# Autodesk Inventor assembly: ForkMechanism_report
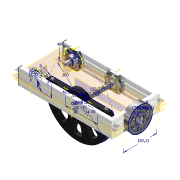
[picture p0: Inventor's stored thumbnail of the model, 180x180]
Saved by Autodesk Inventor 2022 (Build 260153000, 153)
## iProperties
Created: 2022-11-13
Part Number: ForkMechanism_report
Document SubType Name: Assembly
Designer: alexw
Author: alexw
## Documents named in this file (6)
- C:\Users\alexw\Documents\Inventor\Projects\03_CurrentProjects\MasterThesis\PSM_V1_Rillenkugellager\ForkMechanism_report.iam
- C:\Users\alexw\Documents\Inventor\Projects\03_CurrentProjects\MasterThesis\PSM_V1_Rillenkugellager\ParallelMecha_V2_BaseFrame_Item40x40.iam
- C:\Users\alexw\Documents\Inventor\Projects\03_CurrentProjects\MasterThesis\PSM_V1_Rillenkugellager\CapstonDisc_ParallelMecha.ipt
- C:\Users\alexw\Documents\Inventor\Projects\03_CurrentProjects\MasterThesis\PSM_V1_Rillenkugellager\ContentCenter\de-DE\ISO 4762(2)\ISO 4762 - M5 x 16ISO.ipt
- C:\Users\alexw\Documents\Inventor\Projects\03_CurrentProjects\MasterThesis\PSM_V1_Rillenkugellager\ContentCenter\de-DE\ISO 7089\ISO 7089 - 3 - 140 HV(1).ipt
- C:\Users\alexw\Documents\Inventor\Projects\03_CurrentProjects\MasterThesis\PSM_V1_Rillenkugellager\ContentCenter\de-DE\ISO 4762(2)\ISO 4762 - M3 x 8ISO.ipt
## Components (10 placed, 5 different names)
1. ParallelMecha_V2_BaseFrame_Item40x40:1 [sub-assembly]
2. CapstonDisc_ParallelMecha:1 — Passend:13, Passend:15, Passend:16, Passend:19
3. ISO 4762 M5 x 16:1
4. ISO 4762 M5 x 16:2
5. ISO 4762 M5 x 16:3
6. ISO 4762 M5 x 16:4
7. ISO 7089 3:1 — Passend:14
8. ISO 4762 M3 x 8:1 — Passend:13, Passend:14
9. ISO 7089 3:2 — Passend:15, Passend:16, Passend:20
10. ISO 4762 M3 x 8:2 — Passend:19, Passend:20
## Relationships (19: Mate 18, Angle 1)
- [Mate]: ParallelMecha_V2_BaseFrame_Item40x40:1 ↔ CapstonDisc_ParallelMecha:1
- [Mate]: ParallelMecha_V2_BaseFrame_Item40x40:1 ↔ CapstonDisc_ParallelMecha:1
- [Angle] (0 deg): ParallelMecha_V2_BaseFrame_Item40x40:1 ↔ CapstonDisc_ParallelMecha:1
- [Mate]: CapstonDisc_ParallelMecha:1 ↔ ISO 4762 M5 x 16:1
- [Mate]: CapstonDisc_ParallelMecha:1 ↔ ISO 4762 M5 x 16:1
- [Mate]: CapstonDisc_ParallelMecha:1 ↔ ISO 4762 M5 x 16:2
- [Mate]: CapstonDisc_ParallelMecha:1 ↔ ISO 4762 M5 x 16:2
- [Mate]: CapstonDisc_ParallelMecha:1 ↔ ISO 4762 M5 x 16:3
- [Mate]: CapstonDisc_ParallelMecha:1 ↔ ISO 4762 M5 x 16:3
- [Mate]: CapstonDisc_ParallelMecha:1 ↔ ISO 4762 M5 x 16:4
- [Mate]: CapstonDisc_ParallelMecha:1 ↔ ISO 4762 M5 x 16:4
- [Mate]: CapstonDisc_ParallelMecha:1 ↔ ISO 7089 3:1
- [Mate]: CapstonDisc_ParallelMecha:1 ↔ ISO 7089 3:1
- Passend:13 [Mate]: CapstonDisc_ParallelMecha:1 ↔ ISO 4762 M3 x 8:1
- Passend:14 [Mate]: ISO 7089 3:1 ↔ ISO 4762 M3 x 8:1
- Passend:15 [Mate]: CapstonDisc_ParallelMecha:1 ↔ ISO 7089 3:2
- Passend:16 [Mate]: CapstonDisc_ParallelMecha:1 ↔ ISO 7089 3:2
- Passend:19 [Mate]: CapstonDisc_ParallelMecha:1 ↔ ISO 4762 M3 x 8:2
- Passend:20 [Mate]: ISO 7089 3:2 ↔ ISO 4762 M3 x 8:2
